# Autodesk Inventor assembly: 创新设计之指尖积木
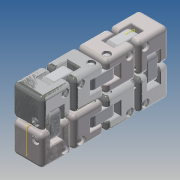
[picture p0: Inventor's stored thumbnail of the model, 180x180]
Saved by Autodesk Inventor 2019.1 (Build 231200000, 200)
## iProperties
Company: 北京理工大学
Created: 2020-10-12
Part Number: 创新设计之指尖积木
Document SubType Name: Assembly
Designer: 谢庆红冰
Author: 谢庆红冰
## Documents named in this file (5)
- F:\学习资料\智能制造实训\unit2\指尖积木_Beta.iam
- F:\学习资料\智能制造实训\unit2\方块1_beta1.ipt
- F:\学习资料\智能制造实训\unit2\方块2_beta.ipt
- F:\学习资料\智能制造实训\unit2\链_beta.ipt
- F:\学习资料\智能制造实训\unit2\轴_bate.ipt
## Components (32 placed, 4 different names)
1. 方块1_beta1:1 — 旋转:1, 刚性:1, 表面齐平:4, 旋转:10, 表面齐平:5, 表面齐平:6, 配合:13, 配合:21
2. 方块2_beta:1 — 旋转:2, 刚性:2, 表面齐平:4, 表面齐平:9, 配合:8, 配合:12, 配合:22, 配合:23
3. 链_beta:1 — 旋转:1, 旋转:2
4. 轴_bate:1 — 刚性:2
5. 轴_bate:2 — 刚性:1
6. 方块1_beta1:2 — 表面齐平:8, 配合:3, 表面齐平:12, 配合:9, 配合:24, 配合:25
7. 方块2_beta:2 — 表面齐平:8, 表面齐平:9, 配合:7, 配合:11, 配合:17
8. 链_beta:2
9. 轴_bate:3
10. 轴_bate:4
11. 方块1_beta1:3 — 表面齐平:7, 配合:6, 表面齐平:12, 配合:10
12. 方块2_beta:3 — 旋转:7, 表面齐平:5, 表面齐平:6, 表面齐平:7, 表面齐平:11, 表面齐平:13, 配合:14, 配合:20
13. 链_beta:3
14. 轴_bate:5
15. 轴_bate:6
16. 链_beta:4 — 旋转:7, 配合:4
17. 链_beta:5 — 旋转:10, 配合:5, 配合:15
18. 链_beta:6 — 配合:7, 配合:8, 配合:17
19. 链_beta:7 — 配合:3, 配合:6
20. 方块1_beta1:4 — 配合:5, 配合:18
21. 方块2_beta:4 — 表面齐平:11, 配合:4, 表面齐平:13, 配合:16, 配合:19
22. 链_beta:8
23. 轴_bate:7
24. 轴_bate:8
25. 轴_bate:9 — 配合:13, 配合:21
26. 轴_bate:10 — 配合:12, 配合:22
27. 轴_bate:11 — 配合:11, 配合:23
28. 轴_bate:12 — 配合:9, 配合:24
29. 轴_bate:13 — 配合:10, 配合:25
30. 轴_bate:14 — 配合:15, 配合:18
31. 轴_bate:15 — 配合:14, 配合:20
32. 轴_bate:16 — 配合:16, 配合:19
## Relationships (51: Mate 23, RevoluteJoint 10, Flush 10, WeldJoint 8)
- 旋转:1 [RevoluteJoint]: 方块1_beta1:1 ↔ 链_beta:1
- 刚性:1 [WeldJoint]: 方块1_beta1:1 ↔ 轴_bate:2
- 旋转:2 [RevoluteJoint]: 方块2_beta:1 ↔ 链_beta:1
- 刚性:2 [WeldJoint]: 方块2_beta:1 ↔ 轴_bate:1
- [RevoluteJoint]: 方块1_beta1:2 ↔ 链_beta:2
- [WeldJoint]: 方块1_beta1:2 ↔ 轴_bate:4
- [RevoluteJoint]: 方块2_beta:2 ↔ 链_beta:2
- [WeldJoint]: 方块2_beta:2 ↔ 轴_bate:3
- [RevoluteJoint]: 方块1_beta1:3 ↔ 链_beta:3
- [WeldJoint]: 方块1_beta1:3 ↔ 轴_bate:6
- [RevoluteJoint]: 方块2_beta:3 ↔ 链_beta:3
- [WeldJoint]: 方块2_beta:3 ↔ 轴_bate:5
- 表面齐平:4 [Flush]: 方块1_beta1:1 ↔ 方块2_beta:1
- 旋转:7 [RevoluteJoint]: 方块2_beta:3 ↔ 链_beta:4
- 旋转:10 [RevoluteJoint]: 方块1_beta1:1 ↔ 链_beta:5
- 表面齐平:5 [Flush]: 方块1_beta1:1 ↔ 方块2_beta:3
- 表面齐平:6 [Flush]: 方块1_beta1:1 ↔ 方块2_beta:3
- 表面齐平:7 [Flush]: 方块1_beta1:3 ↔ 方块2_beta:3
- 表面齐平:8 [Flush]: 方块1_beta1:2 ↔ 方块2_beta:2
- 表面齐平:9 [Flush]: 方块2_beta:1 ↔ 方块2_beta:2
- 配合:3 [Mate]: 方块1_beta1:2 ↔ 链_beta:7
- [RevoluteJoint]: 方块1_beta1:4 ↔ 链_beta:8
- [WeldJoint]: 方块1_beta1:4 ↔ 轴_bate:8
- [RevoluteJoint]: 方块2_beta:4 ↔ 链_beta:8
- [WeldJoint]: 方块2_beta:4 ↔ 轴_bate:7
- [Flush]: 方块1_beta1:4 ↔ 方块2_beta:4
- 表面齐平:11 [Flush]: 方块2_beta:3 ↔ 方块2_beta:4
- 配合:4 [Mate]: 链_beta:4 ↔ 方块2_beta:4
- 配合:5 [Mate]: 链_beta:5 ↔ 方块1_beta1:4
- 配合:6 [Mate]: 方块1_beta1:3 ↔ 链_beta:7
- 配合:7 [Mate]: 方块2_beta:2 ↔ 链_beta:6
- 配合:8 [Mate]: 方块2_beta:1 ↔ 链_beta:6
- 表面齐平:12 [Flush]: 方块1_beta1:2 ↔ 方块1_beta1:3
- 表面齐平:13 [Flush]: 方块2_beta:3 ↔ 方块2_beta:4
- 配合:9 [Mate]: 方块1_beta1:2 ↔ 轴_bate:12
- 配合:10 [Mate]: 方块1_beta1:3 ↔ 轴_bate:13
- 配合:11 [Mate]: 方块2_beta:2 ↔ 轴_bate:11
- 配合:12 [Mate]: 方块2_beta:1 ↔ 轴_bate:10
- 配合:13 [Mate]: 方块1_beta1:1 ↔ 轴_bate:9
- 配合:14 [Mate]: 方块2_beta:3 ↔ 轴_bate:15
- 配合:15 [Mate]: 链_beta:5 ↔ 轴_bate:14
- 配合:16 [Mate]: 方块2_beta:4 ↔ 轴_bate:16
- 配合:17 [Mate]: 方块2_beta:2 ↔ 链_beta:6
- 配合:18 [Mate]: 方块1_beta1:4 ↔ 轴_bate:14
- 配合:19 [Mate]: 方块2_beta:4 ↔ 轴_bate:16
- 配合:20 [Mate]: 方块2_beta:3 ↔ 轴_bate:15
- 配合:21 [Mate]: 方块1_beta1:1 ↔ 轴_bate:9
- 配合:22 [Mate]: 方块2_beta:1 ↔ 轴_bate:10
- 配合:23 [Mate]: 方块2_beta:1 ↔ 轴_bate:11
- 配合:24 [Mate]: 方块1_beta1:2 ↔ 轴_bate:12
- 配合:25 [Mate]: 方块1_beta1:2 ↔ 轴_bate:13
## Named parameters: d7_d2 = 0 mm, d8_d3 = 0 mm, d9_d4 = -90 deg, d10_d5 = 0 mm, d11_d0 = 0 mm, d12_d1 = 90 deg, d14_d2 = 0 mm, d15_d3 = 0 mm, d16_d4 = -90 deg, d17_d5 = 0 mm, d18_d0 = 0 mm, d19_d1 = 90 deg, d50_d45 = 0 mm, d51_d7_d2 = 0 mm, d52_d8_d3 = 0 mm, d53_d9_d4 = -90 deg, d54_d10_d5 = 0 mm, d55_d11_d0 = 0 mm, d56_d12_d1 = 90 deg
